# Autodesk Inventor assembly: Total Assembly v.2
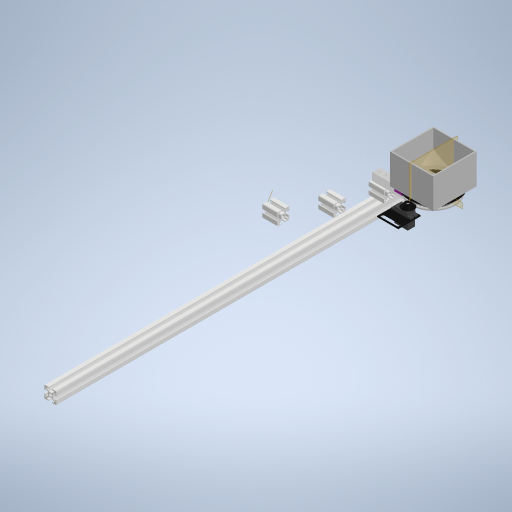
[picture p0: Inventor's stored thumbnail of the model, 512x512]
Saved by Autodesk Inventor 2023 (Build 270158000, 158)
## iProperties
Created: 2022-10-04
Part Number: Total Assembly v.2
Document SubType Name: Assembly
Designer: Raker
Author: Raker
## Documents named in this file (7)
- D:\College Stuff\ATMAE Robotics\Pill Dispenser Robot\Total Assembly Versions\v.2\Total Assembly v.2.iam
- D:\College Stuff\ATMAE Robotics\Pill Dispenser Robot\Frame Stuff\20x20x600 T Slot Extrusion Bar.ipt
- D:\College Stuff\ATMAE Robotics\Pill Dispenser Robot\Frame Stuff\20x20x25 T Slot Extrusion Bar.ipt
- D:\College Stuff\ATMAE Robotics\Pill Dispenser Robot\Threads and Fasteners\T Slot Nut.ipt
- D:\College Stuff\ATMAE Robotics\Pill Dispenser Robot\Load Cell_Hopper_Connection\Load Cell Hopper Interface Designs\v.2\Hopper Interface v.2.iam
- D:\College Stuff\ATMAE Robotics\Pill Dispenser Robot\Hoppers\Hopper Parts\Skittles Hopper Assembly.iam
- D:\College Stuff\ATMAE Robotics\Pill Dispenser Robot\Plates and Brackets\Servo-Bracket Assembly.iam
## Components (8 placed, 6 different names)
1. 20x20x600 T Slot Extrusion Bar:1 — Flush:1, Mate:2, Mate:14, Mate:17
2. 20x20x25 T Slot Extrusion Bar:1 — Mate:1, Mate:2, Mate:4, Mate:5, Mate:12, Mate:13, Mate:14
3. T Slot Nut:1 — Mate:4, Mate:5, Mate:7, Mate:8, Mate:13
4. Hopper Interface v.2:1 [sub-assembly] — Mate:7, Mate:8, Mate:10, Mate:11, Flush:2, Mate:12
5. Skittles Hopper Assembly:1 [sub-assembly] — Mate:10, Mate:11, Flush:2, Mate:15, Mate:16, Flush:3, Tangent:1
6. 20x20x25 T Slot Extrusion Bar:2 — Mate:17
7. 20x20x25 T Slot Extrusion Bar:3
8. Servo-Bracket Assembly:1 [sub-assembly] — Mate:15, Mate:16, Tangent:1
## Relationships (18: Mate 14, Flush 3, Tangent 1)
- Flush:1 (-50 mm): 20x20x600 T Slot Extrusion Bar:1
- Mate:1: 20x20x25 T Slot Extrusion Bar:1
- Mate:2: 20x20x600 T Slot Extrusion Bar:1 ↔ 20x20x25 T Slot Extrusion Bar:1
- Mate:4: 20x20x25 T Slot Extrusion Bar:1 ↔ T Slot Nut:1
- Mate:5: 20x20x25 T Slot Extrusion Bar:1 ↔ T Slot Nut:1
- Mate:7: T Slot Nut:1 ↔ Hopper Interface v.2:1
- Mate:8: T Slot Nut:1 ↔ Hopper Interface v.2:1
- Mate:10: Hopper Interface v.2:1 ↔ Skittles Hopper Assembly:1
- Mate:11: Hopper Interface v.2:1 ↔ Skittles Hopper Assembly:1
- Flush:2: Hopper Interface v.2:1 ↔ Skittles Hopper Assembly:1
- Mate:12: 20x20x25 T Slot Extrusion Bar:1 ↔ Hopper Interface v.2:1
- Mate:13: 20x20x25 T Slot Extrusion Bar:1 ↔ T Slot Nut:1
- Mate:14: 20x20x600 T Slot Extrusion Bar:1 ↔ 20x20x25 T Slot Extrusion Bar:1
- Mate:15: Skittles Hopper Assembly:1 ↔ Servo-Bracket Assembly:1
- Mate:16: Skittles Hopper Assembly:1 ↔ Servo-Bracket Assembly:1
- Flush:3: Skittles Hopper Assembly:1
- Tangent:1: Skittles Hopper Assembly:1 ↔ Servo-Bracket Assembly:1
- Mate:17: 20x20x600 T Slot Extrusion Bar:1 ↔ 20x20x25 T Slot Extrusion Bar:2
